# Autodesk Inventor assembly: Chewbacca
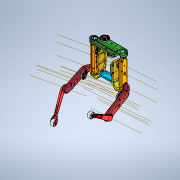
[picture p0: Inventor's stored thumbnail of the model, 180x180]
Saved by Autodesk Inventor 2022.2 (Build 262287000, 287)
## iProperties
Created: 2022-01-14
Part Number: Chewbacca
Document SubType Name: Assembly
Designer: Jochen
Author: Jochen
## Documents named in this file (4)
- D:\Projects\Chewbacca\CAD\Chewbacca.iam
- D:\Projects\Chewbacca\CAD\BodyStructure.iam
- D:\Projects\Chewbacca\CAD\Leg Long.iam
- D:\Projects\Chewbacca\CAD\Leg Short.iam
## Components (3 placed, 3 different names)
1. BodyStructure:1 [sub-assembly] — Mate:1, Mate:2, Mate:3, Mate:4
2. Leg Long:1 [sub-assembly] — Mate:2, Mate:3
3. Leg Short:1 [sub-assembly] — Mate:1, Mate:4
## Relationships (4: Mate 4)
- Mate:1: BodyStructure:1 ↔ Leg Short:1
- Mate:2: BodyStructure:1 ↔ Leg Long:1
- Mate:3: BodyStructure:1 ↔ Leg Long:1
- Mate:4: BodyStructure:1 ↔ Leg Short:1
